# Autodesk Inventor assembly: Montagem1
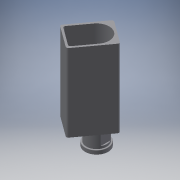
[picture p0: Inventor's stored thumbnail of the model, 180x180]
Saved by Autodesk Inventor 2018 (Build 220112000, 112)
## iProperties
Created: 2018-03-15
Part Number: Montagem1
Material: Genérico
Document SubType Name: Assembly
Designer: Georgines
Author: Georgines
## Documents named in this file (4)
- C:\Users\Georgines\Documents\projeto_estação_bga\Montagem1.iam
- C:\Users\Georgines\Documents\projeto_estação_bga\bocal_de_aquecimento.ipt
- C:\Users\Georgines\Documents\projeto_estação_bga\soprador.ipt
- C:\Users\Georgines\Documents\projeto_estação_bga\carcaça.ipt
## Components (3 placed, 3 different names)
1. bocal_de_aquecimento:1 — Alinhamento:1, Coincidência:1, Alinhamento:2
2. soprador:1 — Alinhamento:1, Coincidência:1, Coincidência:2
3. carcaça:1 — Alinhamento:2, Coincidência:2
## Relationships (4: Flush 2, Mate 2)
- Alinhamento:1 [Flush]: bocal_de_aquecimento:1 ↔ soprador:1
- Coincidência:1 [Mate]: bocal_de_aquecimento:1 ↔ soprador:1
- Alinhamento:2 [Flush]: bocal_de_aquecimento:1 ↔ carcaça:1
- Coincidência:2 [Mate]: soprador:1 ↔ carcaça:1
